# Autodesk Inventor assembly: LEDHolder
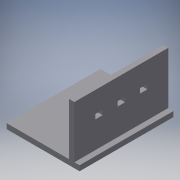
[picture p0: Inventor's stored thumbnail of the model, 180x180]
Saved by Autodesk Inventor 2019 (Build 230136000, 136)
## iProperties
Created: 2018-12-07
Part Number: LEDHolder
Document SubType Name: Assembly
Designer: Administrator
Author: Administrator
## Documents named in this file (3)
- H:\Space\LEDHolder\LEDHolder.iam
- H:\Space\LEDHolder\LEDBottom.ipt
- H:\Space\LEDHolder\LEDFront.ipt
## Components (2 placed, 2 different names)
1. LEDBottom:1 — Mate:1, Flush:1, Flush:2
2. LEDFront:1 — Mate:1, Flush:1, Flush:2
## Relationships (3: Flush 2, Mate 1)
- Mate:1: LEDBottom:1 ↔ LEDFront:1
- Flush:1: LEDBottom:1 ↔ LEDFront:1
- Flush:2: LEDBottom:1 ↔ LEDFront:1
